# Autodesk Inventor assembly: Payload
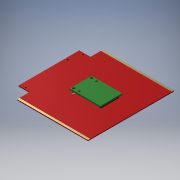
[picture p0: Inventor's stored thumbnail of the model, 180x180]
Saved by Autodesk Inventor 2018 (Build 220112000, 112)
## iProperties
Created: 2018-07-04
Part Number: Payload
Document SubType Name: Assembly
Designer: Bradley
Author: Bradley
## Documents named in this file (3)
- D:\Users\Bradley\Documents\CougsInSpace\CougSat1-Hardware\CougSat1-Payload\CADModel\Native\Payload.iam
- D:\Users\Bradley\Documents\CougsInSpace\CougSat1-Hardware\CougSat1-Payload\CADModel\Native\Payload_PCB.ipt
- D:\Users\Bradley\Documents\CougsInSpace\Resources\ComponentModels\Electronics\Module_ArducamMini-Rev.ipt
## Components (2 placed, 2 different names)
1. Payload_PCB:1 — Mate:1, Mate:3
2. Module_ArducamMini-Rev:1 — Mate:1, Mate:2, Mate:3
## Relationships (3: Mate 3)
- Mate:1: Payload_PCB:1 ↔ Module_ArducamMini-Rev:1
- Mate:2: Module_ArducamMini-Rev:1
- Mate:3: Payload_PCB:1 ↔ Module_ArducamMini-Rev:1
